# Autodesk Inventor assembly: Assembly_base
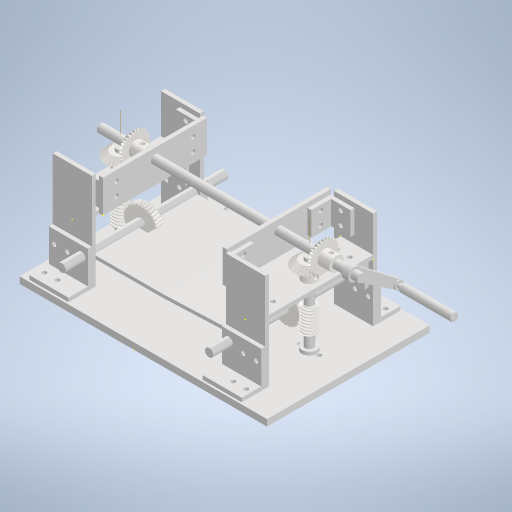
[picture p0: Inventor's stored thumbnail of the model, 512x512]
Saved by Autodesk Inventor 2023 (Build 270158000, 158)
## iProperties
Created: 2023-02-09
Part Number: Assembly_base
Document SubType Name: Assembly
Designer: deepa
Author: deepa
## Documents named in this file (17)
- C:\Users\deepa\OneDrive\Desktop\Courses\4thsem\ta220\Group 27 TA\Assembly_base.iam
- C:\Users\deepa\OneDrive\Desktop\Courses\4thsem\ta220\Group 27 TA\Base Plate.ipt
- C:\Users\deepa\OneDrive\Desktop\Courses\4thsem\ta220\Group 27 TA\Base_Connector1.ipt
- C:\Users\deepa\OneDrive\Desktop\Courses\4thsem\ta220\Group 27 TA\Base_Connector2.ipt
- C:\Users\deepa\OneDrive\Desktop\Courses\4thsem\ta220\Group 27 TA\Side_Plate1.ipt
- C:\Users\deepa\OneDrive\Desktop\Courses\4thsem\ta220\Group 27 TA\Side_plate2.ipt
- C:\Users\deepa\OneDrive\Desktop\Courses\4thsem\ta220\Group 27 TA\support plate 2.ipt
- C:\Users\deepa\OneDrive\Desktop\Courses\4thsem\ta220\Group 27 TA\Normal_Connector.ipt
- C:\Users\deepa\OneDrive\Desktop\Courses\4thsem\ta220\Group 27 TA\support plate 3.ipt
- C:\Users\deepa\OneDrive\Desktop\Courses\4thsem\ta220\Group 27 TA\rod_450mm.ipt
- C:\Users\deepa\OneDrive\Desktop\Courses\4thsem\ta220\Group 27 TA\shaft_120mm.ipt
- C:\Users\deepa\OneDrive\Desktop\Courses\4thsem\ta220\Group 27 TA\Assembly_base\Design Accelerator\Bevel Gears3.iam
- C:\Users\deepa\OneDrive\Desktop\Courses\4thsem\ta220\Group 27 TA\rod_250mm.ipt
- C:\Users\deepa\OneDrive\Desktop\Courses\4thsem\ta220\Group 27 TA\Assembly_base\Design Accelerator\Worm Gears7.iam
- C:\Users\deepa\OneDrive\Desktop\Courses\4thsem\ta220\Group 27 TA\sadak_.ipt
- C:\Users\deepa\OneDrive\Desktop\Courses\4thsem\ta220\Group 27 TA\Handle.ipt
- C:\Users\deepa\OneDrive\Desktop\Courses\4thsem\ta220\Group 27 TA\Handle_holder.ipt
## Components (34 placed, 16 different names)
1. Base Plate:1 — Mate:1, Mate:2, Mate:3, Mate:4, Mate:5, Mate:6, Mate:7, Mate:8, Mate:9, Mate:10, Mate:11, Mate:12, Mate:13, Mate:14, Mate:15, Mate:16, Mate:21, Mate:74, Mate:75, Mate:86, Mate:87, Flush:10
2. Base_Connector1:1 — Mate:1, Mate:2, Mate:3, Mate:22, Mate:23
3. Base_Connector1:2 — Mate:4, Mate:5, Mate:6, Mate:26, Mate:32
4. Base_Connector2:1 — Mate:7, Mate:11, Mate:12, Mate:18, Mate:19, Mate:95
5. Base_Connector2:2 — Mate:8, Mate:9, Mate:10, Mate:24, Mate:25, Mate:92
6. Side_Plate1:1 — Mate:14, Mate:21, Mate:22, Mate:23, Mate:40, Flush:1, Mate:54, Mate:99
7. Side_plate2:1 — Mate:13, Mate:18, Mate:19, Flush:2, Mate:45, Mate:46, Mate:72, Mate:98
8. Side_Plate1:2 — Mate:15, Mate:24, Mate:25, Mate:39, Flush:3, Mate:51
9. Side_plate2:2 — Mate:16, Mate:26, Mate:32, Flush:4, Mate:57
10. support plate 2:1 — Mate:36, Mate:37, Mate:38, Mate:40, Flush:1, Mate:53, Mate:73
11. Normal_Connector:1 — Mate:36, Mate:38, Mate:39, Flush:5
12. Normal_Connector:2 — Mate:37, Mate:54, Flush:6
13. support plate 2:2 — Flush:2, Mate:46, Mate:56, Mate:58
14. Normal_Connector:3 — Mate:45, Flush:6
15. Normal_Connector:4 — Mate:57, Mate:58, Flush:5
16. support plate 3:1 — Flush:4, Mate:56, Mate:61, Mate:62, Mate:69, Mate:70, Mate:71
17. support plate 3:2 — Flush:3, Mate:51, Mate:53, Mate:60, Mate:63, Mate:64, Mate:65, Mate:66, Mate:67, Mate:68
18. Normal_Connector:5 — Mate:66, Mate:67, Mate:68
19. Normal_Connector:6 — Mate:60, Mate:61, Mate:62
20. Normal_Connector:7 — Mate:63, Mate:64, Mate:65
21. Normal_Connector:8 — Mate:69, Mate:70, Mate:71, Mate:72
22. rod_450mm:1 — Mate:73, Flush:10, Mate:88, Mate:90, Mate:100
23. shaft_120mm:1 — Mate:75, Mate:87, Mate:91, Mate:94
24. shaft_120mm:2 — Mate:74, Mate:86, Mate:89, Mate:93
25. Bevel Gears:4 [sub-assembly] — Mate:90, Mate:91, Mate:101
26. Bevel Gears:5 [sub-assembly] — Mate:88, Mate:89
27. rod_250mm:1 — Mate:95, Mate:96
28. rod_250mm:2 — Mate:92, Mate:97
29. Worm Gears:9 [sub-assembly] — Mate:93
30. Worm Gears:10 [sub-assembly] — Mate:94
31. sadak_:1 — Mate:96, Mate:98
32. sadak_:2 — Mate:97, Mate:99
33. Handle:1 — Mate:100, Mate:101, Mate:102, Mate:103
34. Handle_holder:1 — Mate:102, Mate:103
## Relationships (81: Mate 74, Flush 7)
- Mate:1: Base Plate:1 ↔ Base_Connector1:1
- Mate:2: Base Plate:1 ↔ Base_Connector1:1
- Mate:3: Base Plate:1 ↔ Base_Connector1:1
- Mate:4: Base Plate:1 ↔ Base_Connector1:2
- Mate:5: Base Plate:1 ↔ Base_Connector1:2
- Mate:6: Base Plate:1 ↔ Base_Connector1:2
- Mate:7: Base Plate:1 ↔ Base_Connector2:1
- Mate:8: Base Plate:1 ↔ Base_Connector2:2
- Mate:9: Base Plate:1 ↔ Base_Connector2:2
- Mate:10: Base Plate:1 ↔ Base_Connector2:2
- Mate:11: Base Plate:1 ↔ Base_Connector2:1
- Mate:12: Base Plate:1 ↔ Base_Connector2:1
- Mate:13: Base Plate:1 ↔ Side_plate2:1
- Mate:14: Base Plate:1 ↔ Side_Plate1:1
- Mate:15: Base Plate:1 ↔ Side_Plate1:2
- Mate:16: Base Plate:1 ↔ Side_plate2:2
- Mate:18: Base_Connector2:1 ↔ Side_plate2:1
- Mate:19: Base_Connector2:1 ↔ Side_plate2:1
- Mate:21: Base Plate:1 ↔ Side_Plate1:1
- Mate:22: Base_Connector1:1 ↔ Side_Plate1:1
- Mate:23: Base_Connector1:1 ↔ Side_Plate1:1
- Mate:24: Base_Connector2:2 ↔ Side_Plate1:2
- Mate:25: Base_Connector2:2 ↔ Side_Plate1:2
- Mate:26: Base_Connector1:2 ↔ Side_plate2:2
- Mate:32: Base_Connector1:2 ↔ Side_plate2:2
- Mate:36: support plate 2:1 ↔ Normal_Connector:1
- Mate:37: support plate 2:1 ↔ Normal_Connector:2
- Mate:38: support plate 2:1 ↔ Normal_Connector:1
- Mate:39: Side_Plate1:2 ↔ Normal_Connector:1
- Mate:40 (5 mm): Side_Plate1:1 ↔ support plate 2:1
- Flush:1: Side_Plate1:1 ↔ support plate 2:1
- [Mate]: support plate 2:2 ↔ Normal_Connector:3
- [Mate]: support plate 2:2 ↔ Normal_Connector:3
- Flush:2: Side_plate2:1 ↔ support plate 2:2
- Mate:45: Side_plate2:1 ↔ Normal_Connector:3
- Mate:46 (5 mm): Side_plate2:1 ↔ support plate 2:2
- Flush:3: Side_Plate1:2 ↔ support plate 3:2
- Mate:51: Side_Plate1:2 ↔ support plate 3:2
- Mate:53 (10 mm): support plate 2:1 ↔ support plate 3:2
- Mate:54: Side_Plate1:1 ↔ Normal_Connector:2
- Flush:4: Side_plate2:2 ↔ support plate 3:1
- Mate:56 (5 mm): support plate 2:2 ↔ support plate 3:1
- Mate:57: Side_plate2:2 ↔ Normal_Connector:4
- Mate:58: support plate 2:2 ↔ Normal_Connector:4
- Flush:5: Normal_Connector:1 ↔ Normal_Connector:4
- Flush:6: Normal_Connector:2 ↔ Normal_Connector:3
- Mate:60: support plate 3:2 ↔ Normal_Connector:6
- Mate:61: support plate 3:1 ↔ Normal_Connector:6
- Mate:62: support plate 3:1 ↔ Normal_Connector:6
- Mate:63: support plate 3:2 ↔ Normal_Connector:7
- Mate:64: support plate 3:2 ↔ Normal_Connector:7
- Mate:65: support plate 3:2 ↔ Normal_Connector:7
- Mate:66: support plate 3:2 ↔ Normal_Connector:5
- Mate:67: support plate 3:2 ↔ Normal_Connector:5
- Mate:68: support plate 3:2 ↔ Normal_Connector:5
- Mate:69: support plate 3:1 ↔ Normal_Connector:8
- Mate:70: support plate 3:1 ↔ Normal_Connector:8
- Mate:71: support plate 3:1 ↔ Normal_Connector:8
- Mate:72: Side_plate2:1 ↔ Normal_Connector:8
- Mate:73: support plate 2:1 ↔ rod_450mm:1
- Mate:74: Base Plate:1 ↔ shaft_120mm:2
- Mate:75: Base Plate:1 ↔ shaft_120mm:1
- Mate:86: Base Plate:1 ↔ shaft_120mm:2
- Mate:87: Base Plate:1 ↔ shaft_120mm:1
- Flush:10: Base Plate:1 ↔ rod_450mm:1
- Mate:88: rod_450mm:1 ↔ Bevel Gears:5
- Mate:89: shaft_120mm:2 ↔ Bevel Gears:5
- Mate:90: rod_450mm:1 ↔ Bevel Gears:4
- Mate:91: shaft_120mm:1 ↔ Bevel Gears:4
- Mate:92: Base_Connector2:2 ↔ rod_250mm:2
- Mate:93: shaft_120mm:2 ↔ Worm Gears:9
- Mate:94: shaft_120mm:1 ↔ Worm Gears:10
- Mate:95: Base_Connector2:1 ↔ rod_250mm:1
- Mate:96: rod_250mm:1 ↔ sadak_:1
- Mate:97: rod_250mm:2 ↔ sadak_:2
- Mate:98: Side_plate2:1 ↔ sadak_:1
- Mate:99: Side_Plate1:1 ↔ sadak_:2
- Mate:100: rod_450mm:1 ↔ Handle:1
- Mate:101 (20 mm): Bevel Gears:4 ↔ Handle:1
- Mate:102: Handle:1 ↔ Handle_holder:1
- Mate:103: Handle:1 ↔ Handle_holder:1
## Named parameters: d58_d50 = 0 mm, d60_d53 = 0 mm
